# Autodesk Inventor assembly: Drive Base
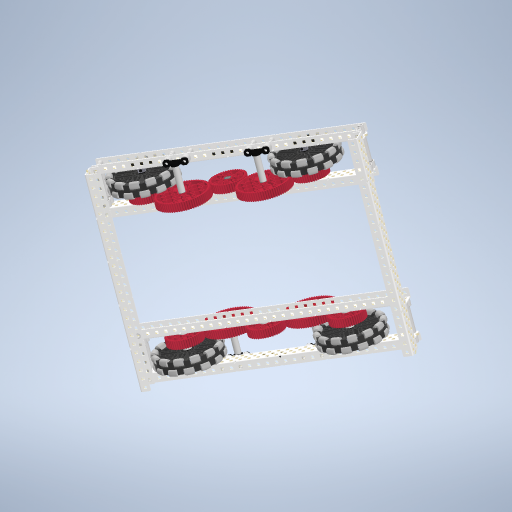
[picture p0: Inventor's stored thumbnail of the model, 512x512]
Saved by Autodesk Inventor 2024 (Build 280153000, 153)
## iProperties
Created: 2023-09-22
Part Number: Drive Base
Document SubType Name: Assembly
Designer: Robodox
Author: Robodox
## Documents named in this file (4)
- C:\Users\Robodox\Documents\GitHub\VEXCAD\Drive Base.iam
- C:\Users\Robodox\Documents\GitHub\VEXCAD\Assembly1.iam
- C:\Users\Robodox\Documents\GitHub\VEXCAD\Part2.ipt
- C:\Users\Robodox\Documents\GitHub\VEX-CAD-Inventor\Structure\C Channel\Aluminum 1x2x1\Alu C 1x2x1x25.ipt
## Components (12 placed, 3 different names)
1. Assembly1:1 [sub-assembly] — Mate:1, Mate:2, Mate:3, Mate:4, Mate:15, Mate:16, Mate:17, Mate:18, Mate:21, Mate:27
2. Part2:1 — Mate:3, Mate:4
3. Part2:2 — Mate:1, Mate:2
4. Part2:3 — Mate:23, Mate:24, Mate:30
5. Part2:4 — Mate:29
6. Part2:5
7. Part2:6 — Mate:22, Mate:25
8. Part2:7 — Mate:15, Mate:18
9. Part2:8 — Mate:16, Mate:17, Mate:21, Mate:26
10. Alu C 1x2x1x25:1 — Mate:23, Mate:24, Mate:26, Flush:2
11. Alu C 1x2x1x25:2 — Mate:22, Mate:25, Mate:27
12. Assembly1:2 [sub-assembly] — Mate:29, Flush:2, Mate:30
## Relationships (18: Mate 17, Flush 1)
- Mate:1: Assembly1:1 ↔ Part2:2
- Mate:2: Assembly1:1 ↔ Part2:2
- Mate:3: Assembly1:1 ↔ Part2:1
- Mate:4: Assembly1:1 ↔ Part2:1
- Mate:15: Assembly1:1 ↔ Part2:7
- Mate:16: Assembly1:1 ↔ Part2:8
- Mate:17: Assembly1:1 ↔ Part2:8
- Mate:18: Assembly1:1 ↔ Part2:7
- Mate:21: Assembly1:1 ↔ Part2:8
- Mate:22: Part2:6 ↔ Alu C 1x2x1x25:2
- Mate:23: Part2:3 ↔ Alu C 1x2x1x25:1
- Mate:24: Part2:3 ↔ Alu C 1x2x1x25:1
- Mate:25: Part2:6 ↔ Alu C 1x2x1x25:2
- Mate:26: Part2:8 ↔ Alu C 1x2x1x25:1
- Mate:27: Assembly1:1 ↔ Alu C 1x2x1x25:2
- Mate:29: Part2:4 ↔ Assembly1:2
- Flush:2: Alu C 1x2x1x25:1 ↔ Assembly1:2
- Mate:30: Part2:3 ↔ Assembly1:2
